# Autodesk Inventor assembly: EixoY
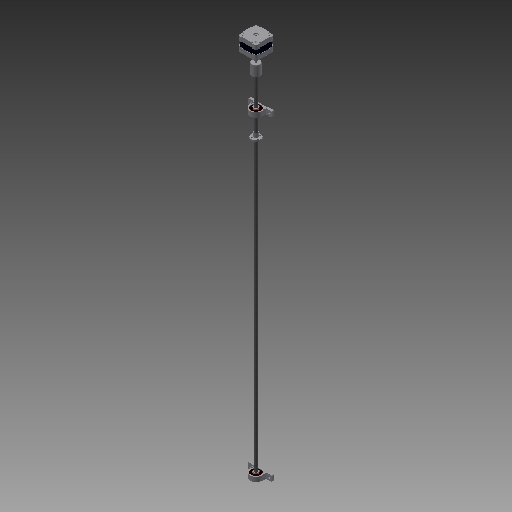
[picture p0: Inventor's stored thumbnail of the model, 512x512]
Saved by Autodesk Inventor 2018 (Build 220112000, 112)
## iProperties
Created: 2018-09-21
Part Number: EixoY
Material: Genérico
Document SubType Name: Assembly
Designer: Georgines
Author: Georgines
## Documents named in this file (6)
- C:\Users\Georgines\Documents\EstacaoBGA\Peças 3D\EixoY.iam
- C:\Users\Georgines\Documents\EstacaoBGA\Peças 3D\kp08.ipt
- C:\Users\Georgines\Documents\EstacaoBGA\Peças 3D\NEMA-17_17HS4401.ipt
- C:\Users\Georgines\Documents\EstacaoBGA\Peças 3D\FusoTrapezoidal_8mmx800mm.ipt
- C:\Users\Georgines\Documents\EstacaoBGA\Peças 3D\Acoplamento5Para8.ipt
- C:\Users\Georgines\Documents\EstacaoBGA\Peças 3D\CastanhaTR8.ipt
## Components (6 placed, 5 different names)
1. kp08:1 — Coincidência:1, Alinhamento:1
2. kp08:2 — Coincidência:2, Alinhamento:2
3. NEMA-17_17HS4401:1 — Inserir:2
4. FusoTrapezoidal_8mmx800mm:1 — Coincidência:1, Alinhamento:1, Coincidência:2, Alinhamento:2, Coincidência:3, Inserir:1
5. Acoplamento5Para8:1 — Inserir:1, Inserir:2
6. CastanhaTR8:1 — Coincidência:3
## Relationships (7: Mate 3, Flush 2, Insert 2)
- Coincidência:1 [Mate]: kp08:1 ↔ FusoTrapezoidal_8mmx800mm:1
- Alinhamento:1 [Flush]: kp08:1 ↔ FusoTrapezoidal_8mmx800mm:1
- Coincidência:2 [Mate]: kp08:2 ↔ FusoTrapezoidal_8mmx800mm:1
- Alinhamento:2 [Flush] (-65 mm): kp08:2 ↔ FusoTrapezoidal_8mmx800mm:1
- Coincidência:3 [Mate]: FusoTrapezoidal_8mmx800mm:1 ↔ CastanhaTR8:1
- Inserir:1: FusoTrapezoidal_8mmx800mm:1 ↔ Acoplamento5Para8:1
- Inserir:2 (-2 mm): NEMA-17_17HS4401:1 ↔ Acoplamento5Para8:1
